# Autodesk Inventor assembly: Gripper_Central_Plate
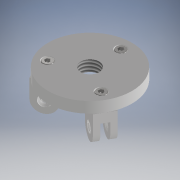
[picture p0: Inventor's stored thumbnail of the model, 180x180]
Saved by Autodesk Inventor 2021.3 (Build 253353000, 353)
## iProperties
Created: 2021-04-16
Part Number: Gripper_Central_Plate
Document SubType Name: Assembly
Designer: domin
Author: domin
## Documents named in this file (4)
- E:\Transfer\Sync\Hivemind\1-MCI-Unterlagen\Master\Semester 2\Projekt 1\Hausberger\Workfolder_Dommy\Gripper\Gripper_Central_Plate.iam
- E:\Transfer\Sync\Hivemind\1-MCI-Unterlagen\Master\Semester 2\Projekt 1\Hausberger\Workfolder_Dommy\Gripper\Gripper_Central_Plate_Base.ipt
- E:\Transfer\Sync\Hivemind\1-MCI-Unterlagen\Master\Semester 2\Projekt 1\Hausberger\Workfolder_Dommy\Gripper\Gripper_Link_Holder.iam
- C:\Users\domin\Documents\Inventor\Content Center Files\R2021\en-US\BS EN ISO 4762\BS EN ISO 4762 - M3 x 8(1).ipt
## Components (7 placed, 3 different names)
1. Gripper_Central_Plate_Base:1 — Mate:1, Mate:2, Mate:3, Mate:4, Mate:7, Mate:9, Mate:11, Mate:13
2. BS EN ISO 4762 - Metric M3 x 8:1 — Mate:8, Mate:9
3. BS EN ISO 4762 - Metric M3 x 8:2 — Mate:10, Mate:11
4. BS EN ISO 4762 - Metric M3 x 8:3 — Mate:12, Mate:13
5. Gripper_Link_Holder:1 [sub-assembly] — Mate:4, Mate:6, Mate:7, Mate:8
6. Gripper_Link_Holder:2 [sub-assembly] — Mate:10
7. Gripper_Link_Holder:3 [sub-assembly] — Mate:12
## Component patterns: (3 elements, first: Gripper_Link_Holder:1)
## Relationships (12: Mate 12)
- Mate:1: Gripper_Central_Plate_Base:1
- Mate:2: Gripper_Central_Plate_Base:1
- Mate:3: Gripper_Central_Plate_Base:1
- Mate:4: Gripper_Central_Plate_Base:1 ↔ Gripper_Link_Holder:1
- Mate:6: Gripper_Link_Holder:1
- Mate:7: Gripper_Central_Plate_Base:1 ↔ Gripper_Link_Holder:1
- Mate:8: BS EN ISO 4762 - Metric M3 x 8:1 ↔ Gripper_Link_Holder:1
- Mate:9: Gripper_Central_Plate_Base:1 ↔ BS EN ISO 4762 - Metric M3 x 8:1
- Mate:10: BS EN ISO 4762 - Metric M3 x 8:2 ↔ Gripper_Link_Holder:2
- Mate:11: Gripper_Central_Plate_Base:1 ↔ BS EN ISO 4762 - Metric M3 x 8:2
- Mate:12: BS EN ISO 4762 - Metric M3 x 8:3 ↔ Gripper_Link_Holder:3
- Mate:13: Gripper_Central_Plate_Base:1 ↔ BS EN ISO 4762 - Metric M3 x 8:3
